# Autodesk Inventor assembly: body
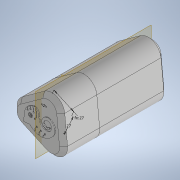
[picture p0: Inventor's stored thumbnail of the model, 180x180]
Saved by Autodesk Inventor 2020 (Build 240168000, 168)
## iProperties
Created: 2019-07-02
Part Number: body
Document SubType Name: Assembly
Designer: erwin
Author: erwin
## Documents named in this file (5)
- D:\GitHub\DrowningWarnings\data_collector\hardware\3x18650_case\body.iam
- D:\GitHub\DrowningWarnings\data_collector\hardware\3x18650_case\case_cap.ipt
- D:\GitHub\DrowningWarnings\data_collector\hardware\3x18650_case\case_bottom.ipt
- D:\GitHub\DrowningWarnings\data_collector\hardware\3x18650_case\body.ipt
- D:\GitHub\DrowningWarnings\data_collector\hardware\3x18650_case\separator.ipt
## Components (3 placed, 3 different names)
1. case_cap:1
2. case_bottom:1 — Flush:1, Flush:2, Flush:3
3. separator:1 — Flush:1, Flush:2
## Relationships (3: Flush 3)
- Flush:1: case_bottom:1 ↔ separator:1
- Flush:2: case_bottom:1 ↔ separator:1
- Flush:3: case_bottom:1
## Named parameters: case_thickness = 2.5 mm
